# Autodesk Inventor assembly: frame
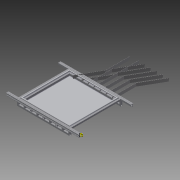
[picture p0: Inventor's stored thumbnail of the model, 180x180]
Saved by Autodesk Inventor 2013 (Build 170138000, 138)
## iProperties
Created: 2012-10-19
Part Number: frame
Document SubType Name: Assembly
Designer: Istvan
Mass: 30866 g
Surface Area: 132817 cm^2
Volume: 17609.3 cm^3
Density: 1.75282 g/cm^3
Author: Istvan
## Documents named in this file (8)
- E:\GitHub\Crown-Fire\CAD\Frame\frame.iam
- E:\GitHub\Crown-Fire\CAD\Frame\Table\table.iam
- E:\GitHub\Crown-Fire\CAD\Frame\Supports\supports.iam
- E:\GitHub\Crown-Fire\CAD\Linear Motion\rack.ipt
- E:\GitHub\Crown-Fire\CAD\GantryMount\cChannel.ipt
- D:\GitHub\Crown-Fire\CAD\Templates\cChannel2x1.ipt
- E:\GitHub\Crown-Fire\CAD\Linear Motion\vee-track.ipt
- E:\GitHub\Crown-Fire\CAD\Linear Motion\vee-track-x.ipt
## Components (8 placed, 6 different names)
1. table:1 [sub-assembly] — Mate:5, Mate:18, Mate:19
2. supports:1 [sub-assembly] — Mate:5, Mate:7, Mate:8, Flush:1, Flush:2, Flush:3, Flush:4, Mate:18, Mate:19
3. rack:1 — Flush:5, Mate:15, Flush:9
4. rack:2 — Flush:6, Mate:14, Flush:10
5. cChannel:1 — Mate:8, Flush:2, Flush:4, Flush:5, Mate:11, Flush:8, Mate:15, Mate:17, Flush:9
6. cChannel:2 — Mate:7, Flush:1, Flush:3, Flush:6, Mate:12, Flush:7, Mate:14, Mate:16, Flush:10
7. vee-track-x:1 — Mate:12, Flush:7, Mate:16
8. vee-track:2 — Mate:11, Flush:8, Mate:17
## Relationships (21: Mate 11, Flush 10)
- Mate:5: table:1 ↔ supports:1
- Mate:7: supports:1 ↔ cChannel:2
- Mate:8: supports:1 ↔ cChannel:1
- Flush:1: supports:1 ↔ cChannel:2
- Flush:2: supports:1 ↔ cChannel:1
- Flush:3: supports:1 ↔ cChannel:2
- Flush:4: supports:1 ↔ cChannel:1
- Flush:5: rack:1 ↔ cChannel:1
- Flush:6: rack:2 ↔ cChannel:2
- Mate:11: cChannel:1 ↔ vee-track:2
- Mate:12: cChannel:2 ↔ vee-track-x:1
- Flush:7: cChannel:2 ↔ vee-track-x:1
- Flush:8: cChannel:1 ↔ vee-track:2
- Mate:14: rack:2 ↔ cChannel:2
- Mate:15: rack:1 ↔ cChannel:1
- Mate:16 (12.7 mm): cChannel:2 ↔ vee-track-x:1
- Mate:17 (12.7 mm): cChannel:1 ↔ vee-track:2
- Mate:18 (12.7 mm): table:1 ↔ supports:1
- Mate:19 (12.7 mm): table:1 ↔ supports:1
- Flush:9 (6.35 mm): rack:1 ↔ cChannel:1
- Flush:10 (6.35 mm): rack:2 ↔ cChannel:2
